# Autodesk Inventor assembly: 部件1
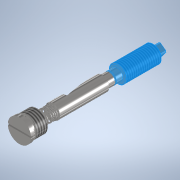
[picture p0: Inventor's stored thumbnail of the model, 180x180]
Saved by Autodesk Inventor 2022 (Build 260153000, 153)
## iProperties
Created: 2023-01-10
Part Number: 部件1
Document SubType Name: Assembly
Designer: Lzy18
Author: Lzy18
## Documents named in this file (5)
- C:\Users\Lzy18\Desktop\夹体\部件1.iam
- C:\Users\Lzy18\Desktop\夹体\9-滑轴.ipt
- C:\Users\Lzy18\Desktop\夹体\2-螺塞.ipt
- C:\Users\Lzy18\Desktop\夹体\Compress Spring11.ipt
- C:\Users\Lzy18\Desktop\夹体\10-螺杆.ipt
## Components (4 placed, 4 different names)
1. 9-滑轴:1 — 配合:4, 配合:5, 配合:7, 配合:8
2. 2-螺塞:1 — 配合:4
3. Compress Spring1:1 — 配合:6, 表面齐平:2
4. 10-螺杆:1 — 配合:7, 配合:8
## Relationships (7: Mate 5, Flush 2)
- 表面齐平:1 [Flush] (17 mm)
- 配合:4 [Mate]: 9-滑轴:1 ↔ 2-螺塞:1
- 配合:5 [Mate] (28 mm): 9-滑轴:1
- 配合:6 [Mate]: Compress Spring1:1
- 表面齐平:2 [Flush]: Compress Spring1:1
- 配合:7 [Mate]: 9-滑轴:1 ↔ 10-螺杆:1
- 配合:8 [Mate]: 9-滑轴:1 ↔ 10-螺杆:1
